# Autodesk Inventor assembly: Jar Jar
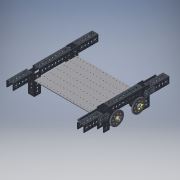
[picture p0: Inventor's stored thumbnail of the model, 180x180]
Saved by Autodesk Inventor 2016 (Build 200138000, 138)
## iProperties
Created: 2015-12-13
Part Number: Jar Jar
Document SubType Name: Assembly
Designer: tbloo
Author: tbloo
## Documents named in this file (9)
- C:\Users\tbloo\Documents\GitHub\phi_robotics\3d-models\FTC_Tetrix_KOP_Block_Party\Tim Bloot Designs\JAr JaR Bot\Jar Jar.iam
- C:\Users\tbloo\Documents\GitHub\phi_robotics\3d-models\FTC_Tetrix_KOP_Block_Party\Tim Bloot Designs\Base Plate.ipt
- C:\Users\tbloo\Documents\GitHub\phi_robotics\3d-models\FTC_Tetrix_KOP_Block_Party\Tim Bloot Designs\JAr JaR Bot\tetrix_angle-144 MM.ipt
- C:\Users\tbloo\Documents\GitHub\phi_robotics\3d-models\FTC_Tetrix_KOP_Block_Party\Tetrix_Kit_FTC\Autodesk Inventor Files\tetrix_c_channel-3.ipt
- C:\Users\tbloo\Documents\GitHub\phi_robotics\3d-models\FTC_Tetrix_KOP_Block_Party\Tetrix_Kit_FTC\Autodesk Inventor Files\tetrix_c_channel-2.ipt
- C:\Users\tbloo\Documents\GitHub\phi_robotics\3d-models\FTC_Tetrix_KOP_Block_Party\Tetrix_Kit_FTC\Autodesk Inventor Files\tetrix_motor_mount-old.ipt
- C:\Users\tbloo\Documents\GitHub\phi_robotics\3d-models\FTC_Tetrix_KOP_Block_Party\Tetrix_Kit_FTC\Autodesk Inventor Files\tetrix_739274_2013.ipt
- C:\Users\tbloo\Documents\GitHub\phi_robotics\3d-models\FTC_Tetrix_KOP_Block_Party\Tetrix_Kit_FTC\Autodesk Inventor Files\tetrix_motor.iam
- C:\Users\tbloo\Documents\GitHub\phi_robotics\3d-models\FTC_Tetrix_KOP_Block_Party\Tim Bloot Designs\JAr JaR Bot\Motor Med Gear.iam
## Components (21 placed, 8 different names)
1. Base Plate:1 — Rigid:1, Rigid:4
2. tetrix_c_channel-3:1
3. tetrix_c_channel-3:2 — Rigid:3, Rigid:5
4. tetrix_c_channel-2:1
5. tetrix_c_channel-2:2 — Rigid:6, Rigid:8, Rigid:10
6. tetrix_c_channel-2:3
7. tetrix_c_channel-2:4 — Rigid:7, Rigid:9, Rigid:12
8. tetrix_c_channel-2:5
9. tetrix_c_channel-2:6
10. tetrix_c_channel-2:7 — Rigid:11
11. tetrix_c_channel-2:8 — Rigid:13
12. tetrix_angle-144 MM:1 — Rigid:1, Rigid:3, Rigid:6
13. tetrix_angle-144 MM:2 — Rigid:4, Rigid:5, Rigid:7
14. tetrix_motor_mount-old:1 — Rigid:9, Rotational:4
15. tetrix_motor_mount-old:2 — Rigid:8, Rotational:3
16. tetrix_739274_2013:1 — Rigid:10, Rigid:11
17. tetrix_739274_2013:2 — Rigid:12, Rigid:13
18. tetrix_motor:1 [sub-assembly] — Rotational:3, Rigid:15
19. tetrix_motor:2 [sub-assembly] — Rotational:4, Rigid:14
20. Motor Med Gear:1 [sub-assembly] — Rigid:14
21. Motor Med Gear:2 [sub-assembly] — Rigid:15
## Relationships (16: WeldJoint 14, RevoluteJoint 2)
- Rigid:1 [WeldJoint]: Base Plate:1 ↔ tetrix_angle-144 MM:1
- Rigid:3 [WeldJoint]: tetrix_c_channel-3:2 ↔ tetrix_angle-144 MM:1
- Rigid:4 [WeldJoint]: Base Plate:1 ↔ tetrix_angle-144 MM:2
- Rigid:5 [WeldJoint]: tetrix_c_channel-3:2 ↔ tetrix_angle-144 MM:2
- Rigid:6 [WeldJoint]: tetrix_c_channel-2:2 ↔ tetrix_angle-144 MM:1
- Rigid:7 [WeldJoint]: tetrix_c_channel-2:4 ↔ tetrix_angle-144 MM:2
- Rigid:8 [WeldJoint]: tetrix_c_channel-2:2 ↔ tetrix_motor_mount-old:2
- Rigid:9 [WeldJoint]: tetrix_c_channel-2:4 ↔ tetrix_motor_mount-old:1
- Rigid:10 [WeldJoint]: tetrix_c_channel-2:2 ↔ tetrix_739274_2013:1
- Rigid:11 [WeldJoint]: tetrix_c_channel-2:7 ↔ tetrix_739274_2013:1
- Rigid:12 [WeldJoint]: tetrix_c_channel-2:4 ↔ tetrix_739274_2013:2
- Rigid:13 [WeldJoint]: tetrix_c_channel-2:8 ↔ tetrix_739274_2013:2
- Rotational:3 [RevoluteJoint]: tetrix_motor_mount-old:2 ↔ tetrix_motor:1
- Rotational:4 [RevoluteJoint]: tetrix_motor_mount-old:1 ↔ tetrix_motor:2
- Rigid:14 [WeldJoint] (-7.5 mm): tetrix_motor:2 ↔ Motor Med Gear:1
- Rigid:15 [WeldJoint] (-7.5 mm): tetrix_motor:1 ↔ Motor Med Gear:2
